# Autodesk Inventor assembly: caliber_truck
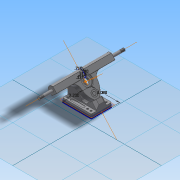
[picture p0: Inventor's stored thumbnail of the model, 180x180]
Saved by Autodesk Inventor 2014 SP2 (Build 180246200, 246)
## iProperties
Created: 2014-02-23
Part Number: caliber_truck
Document SubType Name: Assembly
Designer: Brent Yi
Author: Brent Yi
## Documents named in this file (4)
- C:\Users\dliu\Dropbox\dbhome\electric-longboard\dliu\Mount\Truck Caliber50 9in.iam
- C:\Users\dliu\Dropbox\dbhome\electric-longboard\dliu\Board\Baseplate Caliber50 9in.ipt
- C:\Users\dliu\Dropbox\dbhome\electric-longboard\dliu\Board\Hanger Caliber50 9in.ipt
- C:\Users\dliu\Dropbox\dbhome\electric-longboard\dliu\Board\Generic Riser.ipt
## Components (3 placed, 3 different names)
1. Baseplate Caliber50 9in:1 — Mate:1, Mate:2, TRUCK STRAIGHT Angle:1, Angle:2, Mate:7, Mate:9, Angle:3, Mate:10, Flush:1, Flush:2
2. Hanger Caliber50 9in:1 — Mate:1, Mate:2, TRUCK STRAIGHT Angle:1
3. Generic Riser:1 — Mate:11, Flush:1, Flush:2
## Relationships (11: Mate 6, Angle 3, Flush 2)
- Mate:1: Baseplate Caliber50 9in:1 ↔ Hanger Caliber50 9in:1
- Mate:2: Baseplate Caliber50 9in:1 ↔ Hanger Caliber50 9in:1
- TRUCK STRAIGHT Angle:1 [Angle] (-90 deg): Baseplate Caliber50 9in:1 ↔ Hanger Caliber50 9in:1
- Angle:2 (0 deg): Baseplate Caliber50 9in:1
- Mate:7: Baseplate Caliber50 9in:1
- Mate:9: Baseplate Caliber50 9in:1
- Angle:3 (0 deg): Baseplate Caliber50 9in:1
- Mate:10: Baseplate Caliber50 9in:1
- Mate:11: Generic Riser:1
- Flush:1: Baseplate Caliber50 9in:1 ↔ Generic Riser:1
- Flush:2: Baseplate Caliber50 9in:1 ↔ Generic Riser:1
